# Autodesk Inventor assembly: Assembly146-01
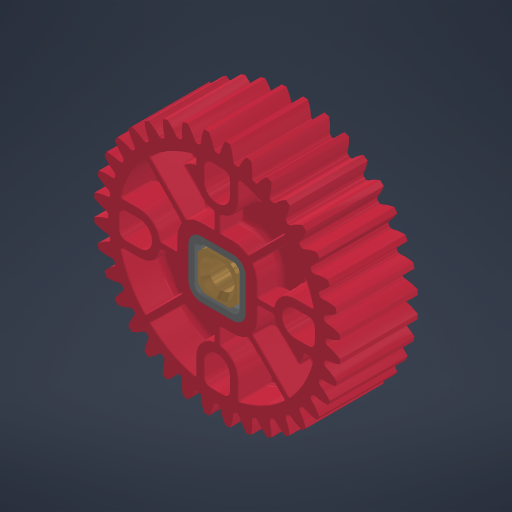
[picture p0: Inventor's stored thumbnail of the model, 512x512]
Saved by Autodesk Inventor 2024 (Build 280153000, 153)
## iProperties
Created: 2022-08-02
Part Number: Assembly146-01
Document SubType Name: Assembly
Designer: ylu12
Author: ylu12
## Documents named in this file (4)
- \\Mac\Home\Desktop\code\1599V-VRC\Cad\Motion\Gears\HS Gear\HS 36T Gear, Circle.iam
- \\Mac\Home\Desktop\code\1599V-VRC\Cad\Motion\HS Shaft Adapter Circle.ipt
- \\Mac\Home\Desktop\code\1599V-VRC\Cad\Motion\Gears\Reference Files\HS 36T Gear, No Insert.ipt
- \\Mac\Home\Desktop\code\1599V-VRC\Cad\Motion\Gears\HS Gear.iam
## Components (2 placed, 2 different names)
1. Circle — Mate:1, Mate:2, Flush:1
2. 36T — Flush:5, Mate:9, Mate:10
## Relationships (6: Mate 4, Flush 2)
- Mate:1: Circle
- Mate:2: Circle
- Flush:1 (6.35 mm): Circle
- Flush:5: 36T
- Mate:9: 36T
- Mate:10: 36T
